# Autodesk Inventor assembly: RobotPallet
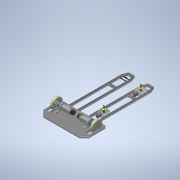
[picture p0: Inventor's stored thumbnail of the model, 180x180]
Saved by Autodesk Inventor 2022.1 (Build 261234000, 234)
## iProperties
Created: 2021-09-10
Part Number: RobotPallet
Material: Generic
Document SubType Name: Assembly
Designer: Andres
Author: Andres
## Documents named in this file (9)
- C:\Users\seb_0\Desktop\PDM\ProyectoRobotPallet\RobotPallet.iam
- C:\Users\seb_0\Desktop\PDM\ProyectoRobotPallet\Estructura Inferior\EstructuraInferior.iam
- C:\Users\seb_0\Desktop\PDM\ProyectoRobotPallet\Estructura Inferior\PlanchaBaseInferior.ipt
- C:\Users\seb_0\Desktop\PDM\ProyectoRobotPallet\SistemaDeElevacion\version2\SistemaElevacionV2.iam
- SistemaElevacion2.iam
- C:\Users\seb_0\Desktop\PDM\ProyectoRobotPallet\Motor\BL Motor + Encoder + Gearbox + Rueda.iam
- C:\Users\seb_0\Desktop\PDM\ProyectoRobotPallet\ContentCenter\es-ES\DIN 630\DIN 630 - 2206 - 30 x 62 x 20.ipt
- C:\Users\seb_0\Desktop\PDM\ProyectoRobotPallet\Soportes\Soporte_Rodamiento.ipt
- C:\Users\seb_0\Desktop\PDM\ProyectoRobotPallet\Soportes\Soporte_Gearbox.ipt
## Components (12 placed, 7 different names)
1. EstructuraInferior:1 [sub-assembly] — Flush:1, Mate:1, Flush:2, Mate:2, Flush:3, Nivelación:4, Nivelación:5, Coincidencia:10, Coincidencia:11, Coincidencia:13, Coincidencia:15, Coincidencia:17, Coincidencia:20
2. PlanchaBaseInferior:1 — Flush:1, Coincidencia:4, Coincidencia:5
3. SistemaElevacion2:1 [sub-assembly] — Mate:1, Flush:2, Mate:3
4. SistemaElevacion2:2 [sub-assembly] — Mate:2, Flush:3, Mate:3
5. BL Motor + Encoder + Gearbox + Rueda:1 [sub-assembly] — Coincidencia:5, Nivelación:5, Coincidencia:9, Nivelación:7, Coincidencia:10, Coincidencia:19, Coincidencia:21
6. BL Motor + Encoder + Gearbox + Rueda:2 [sub-assembly] — Coincidencia:4, Nivelación:4, Coincidencia:8, Nivelación:6, Coincidencia:11, Coincidencia:16, Coincidencia:18
7. DIN 630 2206 - 30 x 62 x 20:1 — Coincidencia:8, Nivelación:6, Coincidencia:14, Nivelación:8
8. DIN 630 2206 - 30 x 62 x 20:2 — Coincidencia:9, Nivelación:7, Coincidencia:12, Nivelación:9
9. Soporte_Rodamiento:1 — Coincidencia:12, Coincidencia:13, Nivelación:9
10. Soporte_Rodamiento:2 — Coincidencia:14, Coincidencia:15, Nivelación:8
11. Soporte_Gearbox:1 — Coincidencia:16, Coincidencia:17, Coincidencia:18
12. Soporte_Gearbox:2 — Coincidencia:19, Coincidencia:20, Coincidencia:21
## Relationships (28: Mate 19, Flush 9)
- Flush:1: EstructuraInferior:1 ↔ PlanchaBaseInferior:1
- Mate:1: EstructuraInferior:1 ↔ SistemaElevacion2:1
- Flush:2: EstructuraInferior:1 ↔ SistemaElevacion2:1
- Mate:2: EstructuraInferior:1 ↔ SistemaElevacion2:2
- Flush:3: EstructuraInferior:1 ↔ SistemaElevacion2:2
- Mate:3 (800 mm): SistemaElevacion2:1 ↔ SistemaElevacion2:2
- Coincidencia:4 [Mate]: PlanchaBaseInferior:1 ↔ BL Motor + Encoder + Gearbox + Rueda:2
- Coincidencia:5 [Mate]: PlanchaBaseInferior:1 ↔ BL Motor + Encoder + Gearbox + Rueda:1
- Nivelación:4 [Flush] (280 mm): EstructuraInferior:1 ↔ BL Motor + Encoder + Gearbox + Rueda:2
- Nivelación:5 [Flush] (280 mm): EstructuraInferior:1 ↔ BL Motor + Encoder + Gearbox + Rueda:1
- Coincidencia:8 [Mate]: BL Motor + Encoder + Gearbox + Rueda:2 ↔ DIN 630 2206 - 30 x 62 x 20:1
- Nivelación:6 [Flush] (-5 mm): BL Motor + Encoder + Gearbox + Rueda:2 ↔ DIN 630 2206 - 30 x 62 x 20:1
- Coincidencia:9 [Mate]: BL Motor + Encoder + Gearbox + Rueda:1 ↔ DIN 630 2206 - 30 x 62 x 20:2
- Nivelación:7 [Flush] (-5 mm): BL Motor + Encoder + Gearbox + Rueda:1 ↔ DIN 630 2206 - 30 x 62 x 20:2
- Coincidencia:10 [Mate] (5 mm): EstructuraInferior:1 ↔ BL Motor + Encoder + Gearbox + Rueda:1
- Coincidencia:11 [Mate] (5 mm): EstructuraInferior:1 ↔ BL Motor + Encoder + Gearbox + Rueda:2
- Coincidencia:12 [Mate]: DIN 630 2206 - 30 x 62 x 20:2 ↔ Soporte_Rodamiento:1
- Coincidencia:13 [Mate]: EstructuraInferior:1 ↔ Soporte_Rodamiento:1
- Coincidencia:14 [Mate]: DIN 630 2206 - 30 x 62 x 20:1 ↔ Soporte_Rodamiento:2
- Coincidencia:15 [Mate]: EstructuraInferior:1 ↔ Soporte_Rodamiento:2
- Nivelación:8 [Flush]: DIN 630 2206 - 30 x 62 x 20:1 ↔ Soporte_Rodamiento:2
- Nivelación:9 [Flush]: DIN 630 2206 - 30 x 62 x 20:2 ↔ Soporte_Rodamiento:1
- Coincidencia:16 [Mate]: BL Motor + Encoder + Gearbox + Rueda:2 ↔ Soporte_Gearbox:1
- Coincidencia:17 [Mate]: EstructuraInferior:1 ↔ Soporte_Gearbox:1
- Coincidencia:18 [Mate] (2.5 mm): BL Motor + Encoder + Gearbox + Rueda:2 ↔ Soporte_Gearbox:1
- Coincidencia:19 [Mate]: BL Motor + Encoder + Gearbox + Rueda:1 ↔ Soporte_Gearbox:2
- Coincidencia:20 [Mate]: EstructuraInferior:1 ↔ Soporte_Gearbox:2
- Coincidencia:21 [Mate] (2.5 mm): BL Motor + Encoder + Gearbox + Rueda:1 ↔ Soporte_Gearbox:2
